# Autodesk Inventor assembly: Main_Assm
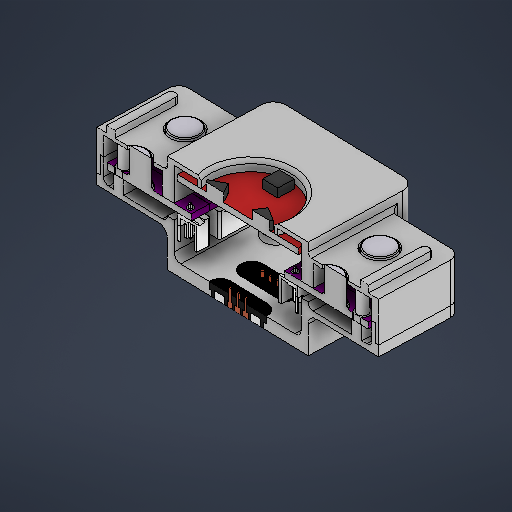
[picture p0: Inventor's stored thumbnail of the model, 512x512]
Saved by Autodesk Inventor 2026 (Build 300175000, 175)
## iProperties
Created: 2025-04-18
Part Number: Main_Assm
Document SubType Name: Assembly
Designer: ct_vi
Author: ct_vi
## Documents named in this file (3)
- C:\Users\ct_vi\Documents\Capstone_Research_3D_Files\Main_Assm.iam
- C:\Users\ct_vi\Documents\Capstone_Research_3D_Files\Main_Top.iam
- C:\Users\ct_vi\Documents\Capstone_Research_3D_Files\Main_Bot.iam
## Components (2 placed, 2 different names)
1. Main_Bot:1 [sub-assembly] — Mate:1, Mate:2, Mate:3
2. Main_Top:1 [sub-assembly] — Mate:1, Mate:2, Mate:3
## Relationships (3: Mate 3)
- Mate:1: Main_Bot:1 ↔ Main_Top:1
- Mate:2: Main_Bot:1 ↔ Main_Top:1
- Mate:3: Main_Bot:1 ↔ Main_Top:1
